# Autodesk Inventor assembly: Robot2
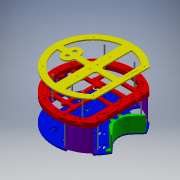
[picture p0: Inventor's stored thumbnail of the model, 180x180]
Saved by Autodesk Inventor 2018.2 (Build 222227000, 227)
## iProperties
Created: 2018-02-26
Part Number: Robot2
Document SubType Name: Assembly
Designer: matth
Mass: 308.249 g
Surface Area: 1876.81 cm^2
Volume: 308.249 cm^3
Density: 1 g/cm^3
Author: matth
## Documents named in this file (8)
- C:\Users\24989\Dropbox\M&A\Robotics-2018\Design and Hardware\mk2\Robot2.iam
- C:\Users\24989\Dropbox\M&A\Robotics-2018\Design and Hardware\mk2\Base\Base3.ipt
- C:\Users\24989\Dropbox\M&A\Robotics-2018\Design and Hardware\mk2\Standoff 20mm.ipt
- C:\Users\24989\Dropbox\M&A\Robotics-2018\Design and Hardware\mk2\Standoff 60mm.ipt
- C:\Users\24989\Dropbox\M&A\Robotics-2018\Design and Hardware\mk2\Tsop Ring-Circuit Board Plate\Tsop Ring-Circuit Board Plate7.ipt
- C:\Users\24989\Dropbox\M&A\Robotics-2018\Design and Hardware\mk2\Wheel Guards\Wheel Guard1.ipt
- C:\Users\24989\Dropbox\M&A\Robotics-2018\Design and Hardware\mk2\Top Plate\Top Plate2.ipt
- C:\Users\24989\Dropbox\M&A\Robotics-2018\Design and Hardware\mk2\Capture Zone\Capture Zone5.ipt
## Components (22 placed, 7 different names)
1. Base3:1 — Mate:4, Mate:5, Mate:6, Mate:7, Mate:8, Mate:9, Mate:10, Mate:17, Mate:18, Mate:19, Mate:20, Mate:21, Mate:30, Mate:31
2. Standoff 60mm:3 — Mate:4
3. Standoff 60mm:4 — Mate:6
4. Standoff 60mm:5 — Mate:10
5. Standoff 60mm:6 — Mate:7, Mate:9
6. Standoff 60mm:7 — Mate:8
7. Standoff 60mm:9 — Mate:5
8. Tsop Ring-Circuit Board Plate7:1 — Mate:16, Mate:25, Mate:26, Mate:27, Mate:28
9. Standoff 20mm:1
10. Standoff 20mm:2 — Mate:16
11. Wheel Guard1:1 — Mate:19, Mate:23
12. Wheel Guard1:2 — Mate:17, Mate:18, Mate:24
13. Wheel Guard1:3 — Mate:20, Mate:21, Mate:22
14. Standoff 20mm:3 — Mate:24
15. Standoff 20mm:4 — Mate:22
16. Standoff 20mm:5 — Mate:23
17. Standoff 60mm:10 — Mate:26
18. Standoff 60mm:11 — Mate:27
19. Standoff 60mm:12 — Mate:28
20. Standoff 60mm:13 — Mate:25, Mate:29
21. Top Plate2:1 — Mate:29
22. Capture Zone5:1 — Mate:30, Mate:31
## Relationships (23: Mate 23)
- Mate:4: Base3:1 ↔ Standoff 60mm:3
- Mate:5: Base3:1 ↔ Standoff 60mm:9
- Mate:6: Base3:1 ↔ Standoff 60mm:4
- Mate:7: Base3:1 ↔ Standoff 60mm:6
- Mate:8: Base3:1 ↔ Standoff 60mm:7
- Mate:9: Base3:1 ↔ Standoff 60mm:6
- Mate:10: Base3:1 ↔ Standoff 60mm:5
- Mate:16: Tsop Ring-Circuit Board Plate7:1 ↔ Standoff 20mm:2
- Mate:17: Base3:1 ↔ Wheel Guard1:2
- Mate:18: Base3:1 ↔ Wheel Guard1:2
- Mate:19: Base3:1 ↔ Wheel Guard1:1
- Mate:20: Base3:1 ↔ Wheel Guard1:3
- Mate:21: Base3:1 ↔ Wheel Guard1:3
- Mate:22: Wheel Guard1:3 ↔ Standoff 20mm:4
- Mate:23: Wheel Guard1:1 ↔ Standoff 20mm:5
- Mate:24: Wheel Guard1:2 ↔ Standoff 20mm:3
- Mate:25: Tsop Ring-Circuit Board Plate7:1 ↔ Standoff 60mm:13
- Mate:26: Tsop Ring-Circuit Board Plate7:1 ↔ Standoff 60mm:10
- Mate:27: Tsop Ring-Circuit Board Plate7:1 ↔ Standoff 60mm:11
- Mate:28: Tsop Ring-Circuit Board Plate7:1 ↔ Standoff 60mm:12
- Mate:29: Standoff 60mm:13 ↔ Top Plate2:1
- Mate:30: Base3:1 ↔ Capture Zone5:1
- Mate:31: Base3:1 ↔ Capture Zone5:1
